# Autodesk Inventor assembly: NoiseSource
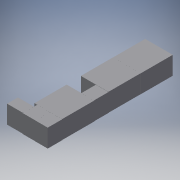
[picture p0: Inventor's stored thumbnail of the model, 180x180]
Saved by Autodesk Inventor 2016 (Build 200138000, 138)
## iProperties
Created: 2016-08-31
Part Number: NoiseSource
Document SubType Name: Assembly
Designer: jfixelle
Author: jfixelle
## Documents named in this file (4)
- E:\jfixelle\Documents\APC\GitRepo\FrontEnd\Placement\NoiseSource.iam
- E:\jfixelle\Documents\APC\GitRepo\FrontEnd\Placement\AmplifierBlock1.ipt
- E:\jfixelle\Documents\APC\GitRepo\FrontEnd\Placement\SwitchBlock.ipt
- E:\jfixelle\Documents\APC\GitRepo\FrontEnd\Placement\UMCCBlock.ipt
## Components (7 placed, 3 different names)
1. AmplifierBlock1:1 — Flush:3
2. SwitchBlock:1 — Flush:2
3. UMCCBlock:1 — Flush:6
4. SwitchBlock:2 — Flush:5
5. SwitchBlock:3 — Flush:4
6. AmplifierBlock1:2 — Flush:1
7. AmplifierBlock1:3 — Flush:1, Flush:2, Flush:3, Flush:4, Flush:5, Flush:6
## Relationships (6: Flush 6)
- Flush:1: AmplifierBlock1:2 ↔ AmplifierBlock1:3
- Flush:2: SwitchBlock:1 ↔ AmplifierBlock1:3
- Flush:3: AmplifierBlock1:1 ↔ AmplifierBlock1:3
- Flush:4: SwitchBlock:3 ↔ AmplifierBlock1:3
- Flush:5: SwitchBlock:2 ↔ AmplifierBlock1:3
- Flush:6: UMCCBlock:1 ↔ AmplifierBlock1:3
